# Autodesk Inventor assembly: Interfaz_I2C
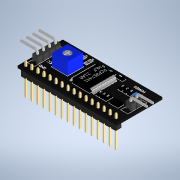
[picture p0: Inventor's stored thumbnail of the model, 180x180]
Saved by Autodesk Inventor 2021 (Build 250183000, 183)
## iProperties
Created: 2022-06-27
Part Number: Interfaz_I2C
Document SubType Name: Assembly
Designer: Tecneu
Author: Tecneu
## Documents named in this file (6)
- C:\Users\Tecneu\Documents\ZD\Modelos 3D\Pantalla LCD + I2C\Interfaz_I2C.iam
- C:\Users\Tecneu\Documents\ZD\Modelos 3D\Pantalla LCD + I2C\Part2_I2C.ipt
- C:\Users\Tecneu\Documents\ZD\Modelos 3D\Pantalla LCD + I2C\1x15 Male Pin Header.ipt
- C:\Users\Tecneu\Documents\ZD\Modelos 3D\Pantalla LCD + I2C\1x1 Male Pin Header.ipt
- C:\Users\Tecneu\Documents\ZD\Modelos 3D\Pantalla LCD + I2C\2Pin.iam
- C:\Users\Tecneu\Documents\ZD\Modelos 3D\Pantalla LCD + I2C\4Pin.iam
## Components (5 placed, 5 different names)
1. Part2_I2C:1 — Flush:1, Flush:2, Flush:3, Mate:2, Mate:3, Mate:4, Mate:5, Flush:6, Flush:7, Flush:8, Flush:9, Mate:6
2. 1x15 Male Pin Header:1 — Flush:4, Mate:1, Flush:5, Mate:4
3. 1x1 Male Pin Header:1 — Flush:4, Mate:1, Flush:5, Mate:2, Mate:3
4. 2Pin:1 [sub-assembly] — Flush:8, Flush:9, Mate:6
5. 4Pin:1 [sub-assembly] — Mate:5, Flush:6, Flush:7
## Relationships (15: Flush 9, Mate 6)
- Flush:1: Part2_I2C:1
- Flush:2: Part2_I2C:1
- Flush:3: Part2_I2C:1
- Flush:4: 1x15 Male Pin Header:1 ↔ 1x1 Male Pin Header:1
- Mate:1: 1x15 Male Pin Header:1 ↔ 1x1 Male Pin Header:1
- Flush:5: 1x15 Male Pin Header:1 ↔ 1x1 Male Pin Header:1
- Mate:2: Part2_I2C:1 ↔ 1x1 Male Pin Header:1
- Mate:3: Part2_I2C:1 ↔ 1x1 Male Pin Header:1
- Mate:4: Part2_I2C:1 ↔ 1x15 Male Pin Header:1
- Mate:5: Part2_I2C:1 ↔ 4Pin:1
- Flush:6 (1.25 mm): Part2_I2C:1 ↔ 4Pin:1
- Flush:7 (4.5 mm): Part2_I2C:1 ↔ 4Pin:1
- Flush:8 (7 mm): Part2_I2C:1 ↔ 2Pin:1
- Flush:9 (1.25 mm): Part2_I2C:1 ↔ 2Pin:1
- Mate:6: Part2_I2C:1 ↔ 2Pin:1
